# Autodesk Inventor assembly: dummy_atx
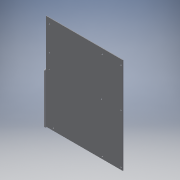
[picture p0: Inventor's stored thumbnail of the model, 180x180]
Saved by Autodesk Inventor 2018 (Build 220112000, 112)
## iProperties
Created: 2021-04-25
Part Number: dummy_atx
Document SubType Name: Assembly
Designer: gisen
Author: gisen
## Documents named in this file (4)
- C:\Users\sbbgi\Documents\GitHub\eatx_case\atx\resources\motherboard\dummy_atx.iam
- C:\Users\sbbgi\Documents\GitHub\eatx_case\atx\resources\motherboard\atxboard.ipt
- C:\Users\sbbgi\Documents\GitHub\eatx_case\atx\resources\motherboard\R5E io shield.ipt
- C:\Users\sbbgi\Documents\GitHub\eatx_case\atx\resources\motherboard\16x.ipt
## Components (5 placed, 3 different names)
1. atxboard:1 — Mate:1, Mate:2, Mate:3, Angle:1, Angle:2, Angle:3, Mate:4, Flush:3, Flush:4
2. R5E io shield:1 — Mate:4, Flush:3, Flush:4
3. 16x:1 — Mate:2, Angle:1, Flush:1
4. 16x:2 — Mate:3, Angle:2, Flush:1, Flush:2
5. 16x:3 — Mate:1, Angle:3, Flush:2
## Relationships (11: Mate 4, Flush 4, Angle 3)
- Mate:1: atxboard:1 ↔ 16x:3
- Mate:2: atxboard:1 ↔ 16x:1
- Mate:3: atxboard:1 ↔ 16x:2
- Angle:1 (0 deg): atxboard:1 ↔ 16x:1
- Angle:2 (0 deg): atxboard:1 ↔ 16x:2
- Angle:3 (0 deg): atxboard:1 ↔ 16x:3
- Flush:1: 16x:1 ↔ 16x:2
- Flush:2: 16x:2 ↔ 16x:3
- Mate:4 (1 mm): atxboard:1 ↔ R5E io shield:1
- Flush:3 (-2.159 mm): atxboard:1 ↔ R5E io shield:1
- Flush:4 (-2.54 mm): atxboard:1 ↔ R5E io shield:1
